# Autodesk Inventor assembly: ensemble
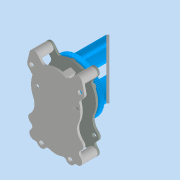
[picture p0: Inventor's stored thumbnail of the model, 180x180]
Saved by Autodesk Inventor 2022 (Build 260153000, 153)
## iProperties
Created: 2022-07-29
Part Number: ensemble
Document SubType Name: Assembly
Designer: andre
Author: andre
## Documents named in this file (6)
- C:\Users\andre\3D Objects\lidar\ensemble.iam
- C:\Users\andre\3D Objects\lidar\top_plate.ipt
- C:\Users\andre\3D Objects\lidar\gear.ipt
- C:\Users\andre\3D Objects\lidar\mirror_holder.ipt
- C:\Users\andre\3D Objects\lidar\gear_top_ring.ipt
- C:\Users\andre\3D Objects\lidar\bottom_plate.ipt
## Components (5 placed, 5 different names)
1. top_plate:1 — Placage:1, Placage:2, Affleurement:2, Affleurement:3
2. gear:1 — Placage:1, Placage:2, Affleurement:1, Placage:3, Placage:4
3. mirror_holder:1 — Affleurement:1, Placage:3, Placage:4
4. gear_top_ring:1 — Affleurement:2
5. bottom_plate:1 — Affleurement:4, Affleurement:5
## Relationships (9: Flush 5, Mate 4)
- Placage:1 [Mate]: top_plate:1 ↔ gear:1
- Placage:2 [Mate]: top_plate:1 ↔ gear:1
- Affleurement:1 [Flush]: gear:1 ↔ mirror_holder:1
- Placage:3 [Mate]: gear:1 ↔ mirror_holder:1
- Placage:4 [Mate]: gear:1 ↔ mirror_holder:1
- Affleurement:2 [Flush]: top_plate:1 ↔ gear_top_ring:1
- Affleurement:3 [Flush] (12 mm): top_plate:1
- Affleurement:4 [Flush]: bottom_plate:1
- Affleurement:5 [Flush]: bottom_plate:1
